# Autodesk Inventor assembly: 2f2
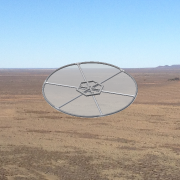
[picture p0: Inventor's stored thumbnail of the model, 180x180]
Saved by Autodesk Inventor 2013 SP2 (Build 170200200, 200)
## iProperties
Company: HERA Project
Created: 2013-06-27
Part Number: 2f2
Document SubType Name: Assembly
Designer: David DeBoer
Description: Feed backplane support assembly
Author: David DeBoer
Title: Feed backplane support
## Documents named in this file (13)
- C:\Users\Dave\Desktop\hera-cad\feed\bpSupAssembly.iam
- C:\Users\Dave\Desktop\hera-cad\feed\bpSupCross.ipt
- C:\Users\Dave\Desktop\hera-cad\feed\bpSupOuter.ipt
- C:\Users\Dave\Desktop\hera-cad\feed\bpSupInner1.ipt
- C:\Users\Dave\Desktop\hera-cad\feed\bpSupInner2.ipt
- C:\Users\Dave\Desktop\hera-cad\feed\collar.ipt
- C:\Users\Dave\Desktop\hera-cad\feed\bpSupArm.ipt
- C:\Users\Dave\Desktop\hera-cad\smallParts\eyebolt_ss_375.ipt
- C:\Users\Dave\Desktop\hera-cad\smallParts\nut_ss_375.ipt
- C:\Users\Dave\Desktop\hera-cad\smallParts\pvc_T_0.75in.ipt
- C:\Users\Dave\Desktop\hera-cad\feed\bpSupArc.ipt
- C:\Users\Dave\Desktop\hera-cad\feed\bpScreen.ipt
- C:\Users\Dave\Desktop\hera-cad\smallParts\D.ipt
## Components (36 placed, 12 different names)
1. bpSupCross:1 — Mate:1, Mate:3, Mate:4, Insert:1, Insert:2, Insert:7
2. collar:1 — Insert:1, Insert:6
3. eyebolt_ss_375:1 — Insert:2, Insert:3
4. nut_ss_375:1 — Insert:3
5. bpScreen:1 — Insert:6
6. bpSupOuter:1 — Mate:1
7. bpSupOuter:2
8. bpSupOuter:3
9. bpSupOuter:4
10. bpSupOuter:5
11. bpSupOuter:6
12. bpSupInner1:2 — Mate:3
13. bpSupInner1:3
14. bpSupInner2:1 — Mate:4
15. bpSupInner2:2
16. bpSupArm:1 — Insert:4
17. bpSupArm:2
18. bpSupArm:3
19. bpSupArm:4
20. bpSupArm:5
21. bpSupArm:6
22. pvc_T_0.75in:1 — Insert:4, Insert:5
23. pvc_T_0.75in:2
24. pvc_T_0.75in:3
25. pvc_T_0.75in:4
26. pvc_T_0.75in:5
27. pvc_T_0.75in:6
28. bpSupArc:1 — Insert:5
29. bpSupArc:2
30. bpSupArc:3
31. bpSupArc:4
32. bpSupArc:5
33. bpSupArc:6
34. D:1 — Insert:7
35. D:2
36. D:3
## Component patterns: outer (6 elements), inner1 (2 elements), inner2 (2 elements), arms (6 elements), Ts (6 elements), (6 elements, first: bpSupArc:1), (3 elements, first: D:1)
## Relationships (10: Insert 7, Mate 3)
- Mate:1: bpSupCross:1 ↔ bpSupOuter:1
- Mate:3: bpSupCross:1 ↔ bpSupInner1:2
- Mate:4: bpSupCross:1 ↔ bpSupInner2:1
- Insert:1: bpSupCross:1 ↔ collar:1
- Insert:2 (-50.8 mm): bpSupCross:1 ↔ eyebolt_ss_375:1
- Insert:3 (-25.4 mm): eyebolt_ss_375:1 ↔ nut_ss_375:1
- Insert:4 (-12.7 mm): bpSupArm:1 ↔ pvc_T_0.75in:1
- Insert:5: pvc_T_0.75in:1 ↔ bpSupArc:1
- Insert:6 (-25.4 mm): collar:1 ↔ bpScreen:1
- Insert:7 (-34.29 mm): bpSupCross:1 ↔ D:1
